# Autodesk Inventor assembly: Assembly
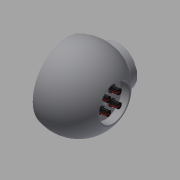
[picture p0: Inventor's stored thumbnail of the model, 180x180]
Saved by Autodesk Inventor 2020 (Build 240168000, 168)
## iProperties
Created: 2020-03-09
Part Number: Assembly
Document SubType Name: Assembly
Designer: user
Author: user
## Documents named in this file (7)
- D:\Documents\Github\Arduino-Smart-light\3DModel\Assembly.iam
- D:\Documents\Github\Arduino-Smart-light\3DModel\Lamp.ipt
- C:\Users\user\Google Drive\Projects\3d\4 Projects\AA Done\.Parts\Potentiometer cap.ipt
- C:\Users\user\Google Drive\Projects\3d\4 Projects\AA Done\.Parts\Potentiometer RV09.ipt
- C:\Users\user\Google Drive\Projects\3d\4 Projects\AA Done\.Parts\Switch TS1233.ipt
- D:\Documents\Github\Arduino-Smart-light\3DModel\PCB.ipt
- C:\Users\user\Google Drive\Projects\3d\4 Projects\AA Done\.Parts\DC jack.ipt
## Components (12 placed, 6 different names)
1. Lamp:1 — Mate:16, Mate:38, Mate:39
2. Potentiometer cap:5 — Flush:4, Flush:6
3. Potentiometer cap:6 — Mate:16, Flush:4, Flush:5
4. Potentiometer cap:7 — Flush:5
5. Potentiometer cap:8 — Flush:6
6. PCB:1 — Mate:26, Mate:27, Mate:28, Mate:29, Mate:30, Mate:31, Mate:32, Mate:36, Mate:37
7. DC jack:1 — Mate:36, Mate:37
8. Switch TS1233:1 — Mate:29, Mate:30, Angle:2
9. Potentiometer RV09:2 — Flush:7, Mate:26, Mate:28, Flush:10, Flush:12, Angle:2, Mate:38, Mate:39
10. Potentiometer RV09:1 — Flush:7, Flush:8, Flush:9, Mate:31, Flush:11, Flush:12
11. Potentiometer RV09:3 — Flush:9, Mate:32, Flush:10, Flush:13
12. Potentiometer RV09:4 — Flush:8, Mate:27, Flush:11, Flush:13
## Relationships (23: Mate 12, Flush 10, Angle 1)
- Mate:16 (0.2 mm): Lamp:1 ↔ Potentiometer cap:6
- Flush:4: Potentiometer cap:5 ↔ Potentiometer cap:6
- Flush:5: Potentiometer cap:6 ↔ Potentiometer cap:7
- Flush:6: Potentiometer cap:5 ↔ Potentiometer cap:8
- Flush:7: Potentiometer RV09:2 ↔ Potentiometer RV09:1
- Flush:8: Potentiometer RV09:1 ↔ Potentiometer RV09:4
- Flush:9: Potentiometer RV09:1 ↔ Potentiometer RV09:3
- Mate:26: PCB:1 ↔ Potentiometer RV09:2
- Mate:27: PCB:1 ↔ Potentiometer RV09:4
- Mate:28: PCB:1 ↔ Potentiometer RV09:2
- Mate:29: PCB:1 ↔ Switch TS1233:1
- Mate:30: PCB:1 ↔ Switch TS1233:1
- Mate:31: PCB:1 ↔ Potentiometer RV09:1
- Mate:32: PCB:1 ↔ Potentiometer RV09:3
- Flush:10: Potentiometer RV09:2 ↔ Potentiometer RV09:3
- Flush:11: Potentiometer RV09:1 ↔ Potentiometer RV09:4
- Flush:12: Potentiometer RV09:2 ↔ Potentiometer RV09:1
- Flush:13: Potentiometer RV09:3 ↔ Potentiometer RV09:4
- Angle:2 (0 deg): Switch TS1233:1 ↔ Potentiometer RV09:2
- Mate:36: PCB:1 ↔ DC jack:1
- Mate:37: PCB:1 ↔ DC jack:1
- Mate:38: Lamp:1 ↔ Potentiometer RV09:2
- Mate:39: Lamp:1 ↔ Potentiometer RV09:2
